# Autodesk Inventor assembly: 2f
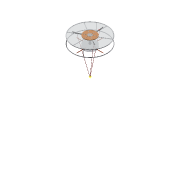
[picture p0: Inventor's stored thumbnail of the model, 180x180]
Saved by Autodesk Inventor 2017 (Build 210142000, 142)
## iProperties
Created: 2013-12-04
Part Number: 2f
Document SubType Name: Assembly
Designer: Dave
Description: Feed assembly
Author: Dave
## Documents named in this file (9)
- C:\Users\krosie\Google Drive\HERA\hera-cad\feed\feedAssembly.iam
- C:\Users\krosie\Google Drive\HERA\hera-cad\feed\bpSupAssembly.iam
- C:\Users\krosie\Google Drive\HERA\hera-cad\feed\dipole.iam
- C:\Users\krosie\Google Drive\HERA\hera-cad\feed\lna.ipt
- C:\Users\krosie\Google Drive\HERA\hera-cad\feed\centralLine.ipt
- C:\Users\krosie\Google Drive\HERA\hera-cad\feed\CentralLine\CentralLine.iam
- C:\Users\krosie\Documents\Inventor\Content Center Files\R2017\en-US\GB 799-88\Eyelet bolt GB 799 M6 x 120.ipt
- C:\Users\krosie\Documents\Inventor\Content Center Files\R2017\en-US\AS 1427(05)\AS 1427 - M6 x 10(5) II.ipt
- C:\Users\krosie\Documents\Inventor\Content Center Files\R2017\en-US\AS 1427(05)\AS 1427 - M5 x 12(5) II.ipt
## Components (15 placed, 8 different names)
1. bpSupAssembly:1 [sub-assembly] — Insert:3, Insert:4, Angle:1, Insert:7, Angle:2, Insert:8, Angle:3, Insert:9, Angle:4, Insert:10, Angle:5
2. dipole:1 [sub-assembly] — Insert:4, Insert:5, Angle:1, Mate:1, Mate:2, Mate:3, Mate:4, Mate:5, Mate:6, Mate:7, Mate:8, Mate:9, Mate:10, Mate:11, Tangent:1, Tangent:2, Tangent:3
3. lna:1 — Insert:5
4. centralLine:1 — Insert:3
5. CentralLine:1 [sub-assembly] — Insert:10, Angle:5
6. Bolt GB/T 799-1988 M6 x 120:4 — Insert:9, Angle:4
7. Bolt GB/T 799-1988 M6 x 120:5 — Insert:8, Angle:3
8. Bolt GB/T 799-1988 M6 x 120:6 — Insert:7, Angle:2
9. AS 1427 H - Metric M6 x 10:1 — Mate:2, Mate:6
10. AS 1427 H - Metric M6 x 10:2 — Mate:1, Mate:7
11. AS 1427 H - Metric M6 x 10:3 — Mate:3, Mate:5
12. AS 1427 H - Metric M6 x 10:4 — Mate:4, Mate:8
13. AS 1427 H - Metric M5 x 12:1 — Mate:10, Tangent:3
14. AS 1427 H - Metric M5 x 12:2 — Mate:9, Tangent:2
15. AS 1427 H - Metric M5 x 12:3 — Mate:11, Tangent:1
## Relationships (26: Mate 11, Insert 7, Angle 5, Tangent 3)
- Insert:3 (25.4 mm): bpSupAssembly:1 ↔ centralLine:1
- Insert:4 (-50.8 mm): bpSupAssembly:1 ↔ dipole:1
- Insert:5 (76.2 mm): dipole:1 ↔ lna:1
- Angle:1 (0 deg): bpSupAssembly:1 ↔ dipole:1
- Insert:7 (-22 mm): bpSupAssembly:1 ↔ Bolt GB/T 799-1988 M6 x 120:6
- Angle:2 (0 deg): bpSupAssembly:1 ↔ Bolt GB/T 799-1988 M6 x 120:6
- Insert:8 (-22 mm): bpSupAssembly:1 ↔ Bolt GB/T 799-1988 M6 x 120:5
- Angle:3 (0 deg): bpSupAssembly:1 ↔ Bolt GB/T 799-1988 M6 x 120:5
- Insert:9 (-22 mm): bpSupAssembly:1 ↔ Bolt GB/T 799-1988 M6 x 120:4
- Angle:4 (0 deg): bpSupAssembly:1 ↔ Bolt GB/T 799-1988 M6 x 120:4
- Insert:10 (1790 mm): bpSupAssembly:1 ↔ CentralLine:1
- Angle:5 (0 deg): bpSupAssembly:1 ↔ CentralLine:1
- Mate:1: dipole:1 ↔ AS 1427 H - Metric M6 x 10:2
- Mate:2: dipole:1 ↔ AS 1427 H - Metric M6 x 10:1
- Mate:3: dipole:1 ↔ AS 1427 H - Metric M6 x 10:3
- Mate:4: dipole:1 ↔ AS 1427 H - Metric M6 x 10:4
- Mate:5: dipole:1 ↔ AS 1427 H - Metric M6 x 10:3
- Mate:6: dipole:1 ↔ AS 1427 H - Metric M6 x 10:1
- Mate:7: dipole:1 ↔ AS 1427 H - Metric M6 x 10:2
- Mate:8: dipole:1 ↔ AS 1427 H - Metric M6 x 10:4
- Mate:9: dipole:1 ↔ AS 1427 H - Metric M5 x 12:2
- Mate:10: dipole:1 ↔ AS 1427 H - Metric M5 x 12:1
- Mate:11: dipole:1 ↔ AS 1427 H - Metric M5 x 12:3
- Tangent:1: dipole:1 ↔ AS 1427 H - Metric M5 x 12:3
- Tangent:2: dipole:1 ↔ AS 1427 H - Metric M5 x 12:2
- Tangent:3: dipole:1 ↔ AS 1427 H - Metric M5 x 12:1
